# Autodesk Inventor assembly: controller
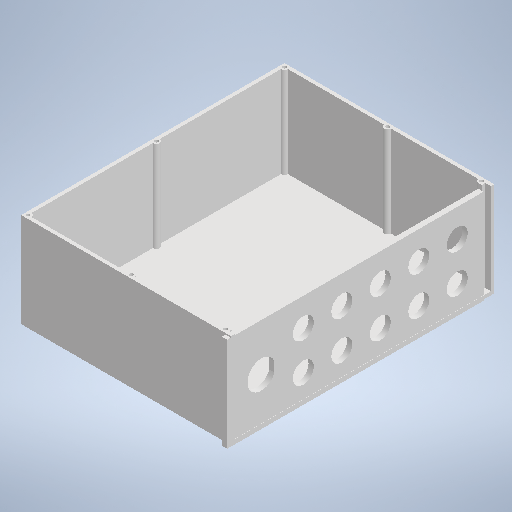
[picture p0: Inventor's stored thumbnail of the model, 512x512]
Saved by Autodesk Inventor 2025.2 (Build 292293000, 293)
## iProperties
Created: 2025-04-21
Part Number: controller
Document SubType Name: Assembly
Designer: tdeboutte
Author: tdeboutte
## Documents named in this file (3)
- C:\Users\tdeboutte\Documents\Projects\bluesmobile\CAD\controller.iam
- C:\Users\tdeboutte\Documents\Projects\bluesmobile\CAD\button-front.ipt
- C:\Users\tdeboutte\Documents\Projects\bluesmobile\CAD\controller-base.ipt
## Components (2 placed, 2 different names)
1. button-front:1 — Mate:1, Mate:2
2. controller-base:1 — Mate:1, Mate:2
## Relationships (2: Mate 2)
- Mate:1: button-front:1 ↔ controller-base:1
- Mate:2: button-front:1 ↔ controller-base:1
